# Autodesk Inventor assembly: Outer_Tube_Adjst_Asm
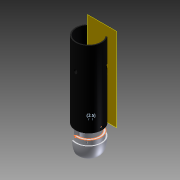
[picture p0: Inventor's stored thumbnail of the model, 180x180]
Saved by Autodesk Inventor 2011 SP2 (Build 150309200, 309)
## iProperties
Created: 2012-06-08
Part Number: Outer_Tube_Adjst_Asm
Document SubType Name: Assembly
Designer: sungwook
Author: sungwook
## Documents named in this file (3)
- C:\Users\sungwook\Documents\Inventor\Micron20_Base_Tube_Adjst\Outer_Tube_Adjst_Asm.iam
- C:\Users\sungwook\Documents\Inventor\Micron20_Base_Tube_Adjst\Outer_Tube.ipt
- C:\Users\sungwook\Documents\Inventor\Micron20_Base_Tube_Adjst\Parts\Handle\Ver2(Al_RP)\Handle_2_Back_rev2.ipt
## Components (2 placed, 2 different names)
1. Outer_Tube:1 — Mate:1, Mate:2
2. Handle_2_Back_rev2:1 — Mate:1, Mate:2
## Relationships (2: Mate 2)
- Mate:1: Outer_Tube:1 ↔ Handle_2_Back_rev2:1
- Mate:2: Outer_Tube:1 ↔ Handle_2_Back_rev2:1
